# Autodesk Inventor assembly: KOP Drive Base D
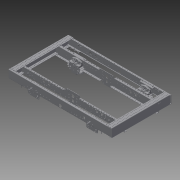
[picture p0: Inventor's stored thumbnail of the model, 180x180]
Saved by Autodesk Inventor 2015 (Build 190159000, 159)
## iProperties
Created: 2015-01-10
Part Number: KOP Drive Base D
Document SubType Name: Assembly
Designer: whitaus15
Title: AM14U2 Long.STEP
Description: STEP AP203
Creation Date: 2014-12-11
Sending System: SolidWorks 2014
Preprocessor: SwSTEP 2.0
Author: whitaus15
## Documents named in this file (7)
- \\lhssvr02\Homedirs\Robotics Club\CAD Model 2015\KOP Drive Base D.iam
- \\lhssvr02\Homedirs\Robotics Club\CAD Model 2015\Imported Components\AM14U2 Long\AM14U2 Half Long.iam
- \\lhssvr02\Homedirs\Robotics Club\CAD Model 2015\Parts Folder\Gear Boxes\Toughbox-mini_MIR6.iam
- \\lhssvr02\Homedirs\Robotics Club\CAD Model 2015\Parts Folder\Gear Boxes\Toughbox-mini_MIR7.iam
- \\lhssvr02\Homedirs\Robotics Club\CAD Model 2015\Parts Folder\Gear Boxes\Toughbox-mini_MIR6_MIR.iam
- \\lhssvr02\Homedirs\Robotics Club\CAD Model 2015\Parts Folder\Gear Boxes\Toughbox-mini_MIR7_MIR.iam
- \\lhssvr02\Homedirs\Robotics Club\CAD Model 2015\Parts Folder\Gear Boxes\Toughbox-mini_MIR6_MIR_MIR.iam
## Components (7 placed, 7 different names)
1. AM14U2 Half Long_1 [sub-assembly] — Symmetry:1, Symmetry:2, Flush:1
2. AM14U2 Half Long_2 [sub-assembly] — Symmetry:1, Symmetry:2, Mate:2, Mate:3, Flush:1
3. Toughbox-mini_MIR6:1 [sub-assembly]
4. Toughbox-mini_MIR7:1 [sub-assembly]
5. Toughbox-mini_MIR6_MIR:1 [sub-assembly]
6. Toughbox-mini_MIR7_MIR:1 [sub-assembly]
7. Toughbox-mini_MIR6_MIR_MIR:1 [sub-assembly] — Mate:2, Mate:3
## Relationships (5: Symmetry 2, Mate 2, Flush 1)
- Symmetry:1: AM14U2 Half Long_1 ↔ AM14U2 Half Long_2
- Symmetry:2: AM14U2 Half Long_1 ↔ AM14U2 Half Long_2
- Mate:2: AM14U2 Half Long_2 ↔ Toughbox-mini_MIR6_MIR_MIR:1
- Mate:3: AM14U2 Half Long_2 ↔ Toughbox-mini_MIR6_MIR_MIR:1
- Flush:1: AM14U2 Half Long_1 ↔ AM14U2 Half Long_2
